# Autodesk Inventor assembly: mascon-new
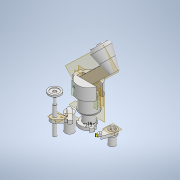
[picture p0: Inventor's stored thumbnail of the model, 180x180]
Saved by Autodesk Inventor 2022 (Build 260153000, 153)
## iProperties
Created: 2021-04-28
Part Number: mascon-new
Document SubType Name: Assembly
Designer: ben
Author: ben
## Documents named in this file (11)
- C:\Users\teh18\OneDrive\BVE Controller\r68-bve-mascon\mascon-new.iam
- C:\Users\teh18\OneDrive\BVE Controller\r68-bve-mascon\handle\handle.iam
- C:\Users\teh18\OneDrive\BVE Controller\r68-bve-mascon\shell\shell.iam
- C:\Users\teh18\OneDrive\BVE Controller\r68-bve-mascon\handle_base_rod.ipt
- C:\Users\teh18\OneDrive\BVE Controller\r68-bve-mascon\handle_holder.ipt
- C:\Users\teh18\OneDrive\BVE Controller\r68-bve-mascon\Reverser.ipt
- C:\Users\teh18\OneDrive\BVE Controller\r68-bve-mascon\reverser-base.ipt
- C:\Users\teh18\OneDrive\BVE Controller\r68-bve-mascon\NotchClickerAsm.iam
- C:\Users\teh18\OneDrive\BVE Controller\r68-bve-mascon\ReverserNotch\ReverserClickAsm.iam
- C:\Users\teh18\OneDrive\BVE Controller\r68-bve-mascon\handle-base\handle_base.iam
- C:\Users\teh18\OneDrive\BVE Controller\r68-bve-mascon\handle_base2.ipt
## Components (10 placed, 10 different names)
1. shell:1 [sub-assembly] — Flush:4, Mate:14, Mate:15, Rotational:2, Flush:15, Mate:22
2. handle_base_rod:1 — Flush:11
3. handle_holder:1 — Mate:16
4. Reverser:1 — Flush:4, Flush:5
5. reverser-base:1 — Flush:5, Flush:6, Flush:10
6. NotchClickerAsm:1 [sub-assembly] — Flush:15, Mate:22
7. ReverserClickAsm:1 [sub-assembly] — Flush:14
8. handle:1 [sub-assembly] — Mate:17, Flush:12, Flush:13, Handle Pop
9. handle_base:1 [sub-assembly] — Mate:14, Mate:15, Mate:16, Mate:17, Rotational:2, Mate:18, Flush:8, Mate:19, Flush:11, Flush:12, Flush:13, Handle Pop
10. handle_base2:1 — Mate:18, Flush:8, Mate:19, Flush:14
## Relationships (19: Flush 10, Mate 7, RevoluteJoint 2)
- Flush:4: shell:1 ↔ Reverser:1
- Flush:5: Reverser:1 ↔ reverser-base:1
- Flush:6 (-36.375 mm): reverser-base:1
- Mate:14: shell:1 ↔ handle_base:1
- Mate:15: shell:1 ↔ handle_base:1
- Mate:16: handle_holder:1 ↔ handle_base:1
- Mate:17: handle:1 ↔ handle_base:1
- Rotational:2 [RevoluteJoint] (-5 mm): shell:1 ↔ handle_base:1
- Mate:18: handle_base:1 ↔ handle_base2:1
- Flush:8: handle_base:1 ↔ handle_base2:1
- Mate:19: handle_base:1 ↔ handle_base2:1
- Flush:10: reverser-base:1
- Flush:11: handle_base_rod:1 ↔ handle_base:1
- Flush:12: handle:1 ↔ handle_base:1
- Flush:13: handle:1 ↔ handle_base:1
- Handle Pop [RevoluteJoint]: handle:1 ↔ handle_base:1
- Flush:14: ReverserClickAsm:1 ↔ handle_base2:1
- Flush:15: shell:1 ↔ NotchClickerAsm:1
- Mate:22: shell:1 ↔ NotchClickerAsm:1
